# Autodesk Inventor assembly: !odom_pod
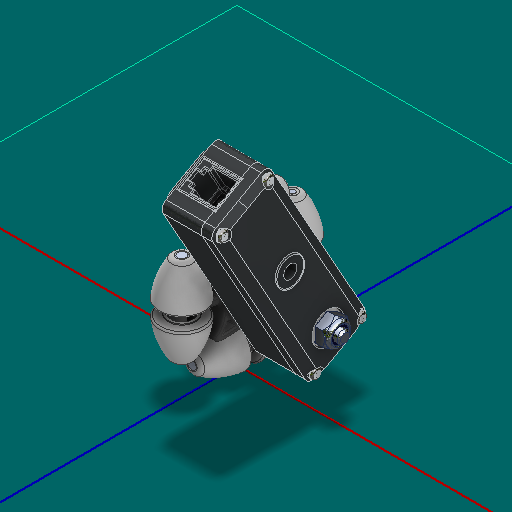
[picture p0: Inventor's stored thumbnail of the model, 512x512]
Saved by Autodesk Inventor 2025 (Build 290162000, 162)
## iProperties
Created: 2024-08-18
Part Number: !odom_pod
Document SubType Name: Assembly
Designer: averey
Author: averey
## Documents named in this file (10)
- C:\Users\avere\vex_robotics_high_stakes\hardware\cad\ATLAS\chassis\odom_pod\!odom_pod.iam
- C:\Users\avere\vex_robotics_high_stakes\hardware\cad\VEX-CAD-Inventor\Motion\Wheels\Omni Wheel\2.00 Omni AS, No Insert.ipt
- C:\Users\avere\vex_robotics_high_stakes\hardware\cad\VEX-CAD-Inventor\Electronics\Sensors\V5 Rotation Sensor.ipt
- C:\Users\avere\vex_robotics_high_stakes\hardware\cad\VEX-CAD-Inventor\Motion\Shaft HS\HS Spacer.ipt
- C:\Users\avere\vex_robotics_high_stakes\hardware\cad\VEX-CAD-Inventor\Motion\Insert Circle.ipt
- C:\Users\avere\vex_robotics_high_stakes\hardware\cad\VEX-CAD-Inventor\Motion\HS Shaft Adapter Circle.ipt
- C:\Users\avere\vex_robotics_high_stakes\hardware\cad\VEX-CAD-Inventor\Motion\Shaft HS\HS Spacer\HSpacer .0625.ipt
- C:\Users\avere\vex_robotics_high_stakes\hardware\cad\VEX-CAD-Inventor\Structure\Hardware\Screw Steel - Star\SScrew Star Smooth 1.750.ipt
- C:\Users\avere\vex_robotics_high_stakes\hardware\cad\VEX-CAD-Inventor\Structure\Hardware\Screw Steel - Star.ipt
- C:\Users\avere\vex_robotics_high_stakes\hardware\cad\VEX-CAD-Inventor\Structure\Hardware\Nut Thin Nylock.ipt
## Components (9 placed, 7 different names)
1. 2.00 Omni AS, No Insert:1 — Insert:1, Angle:1, Angle:4, Insert:5, Angle:5, Insert:9
2. V5 Rotation Sensor:1 — Insert:1, Angle:1, Insert:6
3. Insert Circle:1 — Angle:4, Insert:5, Insert:8, Insert:10
4. Insert Circle:2 — Insert:6, Insert:11
5. HS Shaft Adapter Circle:1 — Insert:7, Flush:1, Angle:5
6. HS Shaft Adapter Circle:2 — Insert:7, Flush:1, Insert:8
7. HSpacer .0625:1 — Insert:9
8. SScrew Star Smooth 1.750:1 — Insert:10
9. Nut Thin Nylock:1 — Insert:11
## Relationships (12: Insert 8, Angle 3, Flush 1)
- Insert:1 (1.5875 mm): 2.00 Omni AS, No Insert:1 ↔ V5 Rotation Sensor:1
- Angle:1 (0 deg): 2.00 Omni AS, No Insert:1 ↔ V5 Rotation Sensor:1
- Angle:4 (0 deg): 2.00 Omni AS, No Insert:1 ↔ Insert Circle:1
- Insert:5: 2.00 Omni AS, No Insert:1 ↔ Insert Circle:1
- Insert:6: V5 Rotation Sensor:1 ↔ Insert Circle:2
- Insert:7: HS Shaft Adapter Circle:1 ↔ HS Shaft Adapter Circle:2
- Flush:1: HS Shaft Adapter Circle:1 ↔ HS Shaft Adapter Circle:2
- Insert:8: Insert Circle:1 ↔ HS Shaft Adapter Circle:2
- Angle:5 (0 deg): 2.00 Omni AS, No Insert:1 ↔ HS Shaft Adapter Circle:1
- Insert:9: 2.00 Omni AS, No Insert:1 ↔ HSpacer .0625:1
- Insert:10: Insert Circle:1 ↔ SScrew Star Smooth 1.750:1
- Insert:11: Insert Circle:2 ↔ Nut Thin Nylock:1
